# Autodesk Inventor assembly: Camera Mount
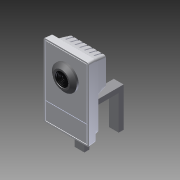
[picture p0: Inventor's stored thumbnail of the model, 180x180]
Saved by Autodesk Inventor 2014 (Build 180170000, 170)
## iProperties
Created: 2014-01-20
Part Number: Camera Mount
Document SubType Name: Assembly
Designer: Andrew Toennies
Author: Andrew Toennies
## Documents named in this file (3)
- C:\Users\Andrew Toennies\Documents\GitHub\2014buildCAD\New Shooter\Camera Mount.iam
- C:\Users\Andrew Toennies\Documents\GitHub\2014buildCAD\New Shooter\Camera Mount.ipt
- C:\Users\Andrew Toennies\Documents\GitHub\2014buildCAD\New Shooter\AXIS-M1011 Camera.ipt
## Components (2 placed, 2 different names)
1. Camera Mount:1 — Mate:1, Mate:2, Mate:3
2. AXIS-M1011 Camera:1 — Mate:1, Mate:2, Mate:3
## Relationships (3: Mate 3)
- Mate:1: Camera Mount:1 ↔ AXIS-M1011 Camera:1
- Mate:2 (18.542 mm): Camera Mount:1 ↔ AXIS-M1011 Camera:1
- Mate:3 (-25.4 mm): Camera Mount:1 ↔ AXIS-M1011 Camera:1
